# Autodesk Inventor assembly: Camera Mold
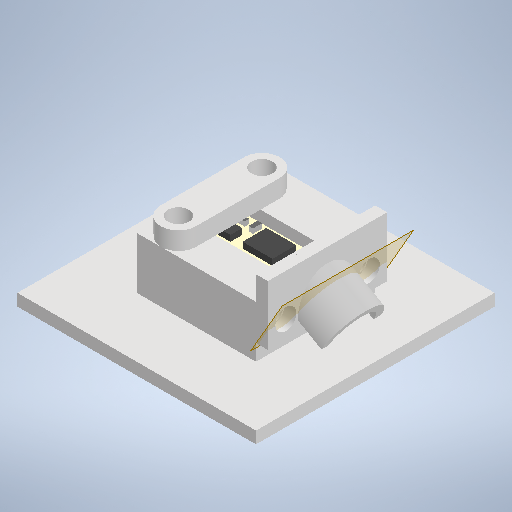
[picture p0: Inventor's stored thumbnail of the model, 512x512]
Saved by Autodesk Inventor 2026.2 (Build 302298010, 298A)
## iProperties
Created: 2026-05-02
Part Number: Camera Mold
Document SubType Name: Assembly
Designer: piete
Author: piete
## Documents named in this file (5)
- C:\Users\piete\Desktop\Skripsie\Documents\Detail Design\Building Parts\Camera Mold.iam
- C:\Users\piete\Desktop\Skripsie\Documents\Detail Design\Micro Robotics Camera Module\Camera assembly.iam
- C:\Users\piete\Desktop\Skripsie\Documents\Detail Design\Building Parts\Camera Holder 1.ipt
- C:\Users\piete\Desktop\Skripsie\Documents\Detail Design\Building Parts\Top Bracket.ipt
- C:\Users\piete\Desktop\Skripsie\Documents\Detail Design\Building Parts\Front Bracket.ipt
## Components (4 placed, 4 different names)
1. Camera assembly:1 [sub-assembly] — Mate:1, Flush:1
2. Camera Holder 1:1 — Mate:1, Flush:1, Mate:2, Mate:3, Mate:4, Mate:5, Mate:6, Mate:7
3. Top Bracket:1 — Mate:2, Mate:3, Mate:4
4. Front Bracket:1 — Mate:5, Mate:6, Mate:7
## Relationships (8: Mate 7, Flush 1)
- Mate:1 (0.25 mm): Camera assembly:1 ↔ Camera Holder 1:1
- Flush:1: Camera assembly:1 ↔ Camera Holder 1:1
- Mate:2: Camera Holder 1:1 ↔ Top Bracket:1
- Mate:3: Camera Holder 1:1 ↔ Top Bracket:1
- Mate:4: Camera Holder 1:1 ↔ Top Bracket:1
- Mate:5: Camera Holder 1:1 ↔ Front Bracket:1
- Mate:6: Camera Holder 1:1 ↔ Front Bracket:1
- Mate:7: Camera Holder 1:1 ↔ Front Bracket:1
